# Autodesk Inventor assembly: 000100
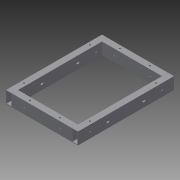
[picture p0: Inventor's stored thumbnail of the model, 180x180]
Saved by Autodesk Inventor 2015 (Build 190159000, 159)
## iProperties
Created: 2015-05-18
Part Number: 000100
Document SubType Name: Assembly
Designer: Wesley
Author: Wesley
## Documents named in this file (3)
- C:\Users\Wesley\Documents\GitHub\EngineeringFinal\Engineering\Engineering Documentation\CADS\0001__\000100.iam
- C:\Users\Wesley\Documents\GitHub\EngineeringFinal\Engineering\Engineering Documentation\CADS\0001__\000101-1.ipt
- C:\Users\Wesley\Documents\GitHub\EngineeringFinal\Engineering\Engineering Documentation\CADS\0001__\000101-2.ipt
## Components (4 placed, 2 different names)
1. 000101-1:1 — Mate:1, Flush:1, Flush:2, Flush:6, Mate:3
2. 000101-2:1 — Mate:1, Flush:1, Flush:2, Mate:2, Flush:3, Flush:4
3. 000101-1:2 — Mate:2, Flush:3, Flush:4, Flush:7
4. 000101-2:2 — Flush:6, Mate:3, Flush:7
## Relationships (9: Flush 6, Mate 3)
- Mate:1: 000101-1:1 ↔ 000101-2:1
- Flush:1: 000101-1:1 ↔ 000101-2:1
- Flush:2: 000101-1:1 ↔ 000101-2:1
- Mate:2: 000101-2:1 ↔ 000101-1:2
- Flush:3: 000101-2:1 ↔ 000101-1:2
- Flush:4: 000101-2:1 ↔ 000101-1:2
- Flush:6: 000101-1:1 ↔ 000101-2:2
- Mate:3: 000101-1:1 ↔ 000101-2:2
- Flush:7: 000101-1:2 ↔ 000101-2:2
